# Autodesk Inventor assembly: Assembly1
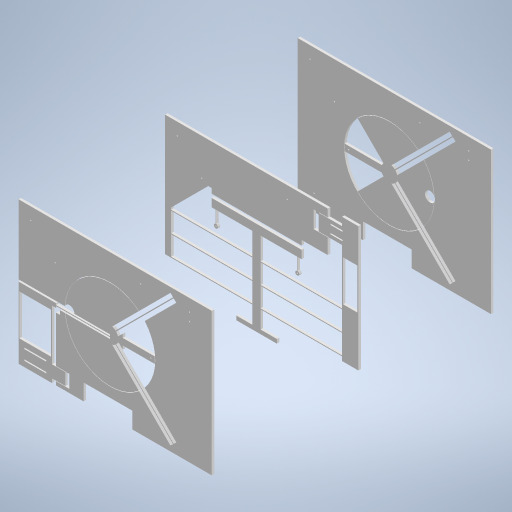
[picture p0: Inventor's stored thumbnail of the model, 512x512]
Saved by Autodesk Inventor 2023 (Build 270158000, 158)
## iProperties
Created: 2023-05-10
Part Number: Assembly1
Document SubType Name: Assembly
Designer: Nathann
Author: Nathann
## Documents named in this file (4)
- C:\Users\Nathann\OneDrive\ClawdDrive\Objet3D\IminaProbe\RoueMDF\Assembly1.iam
- C:\Users\Nathann\OneDrive\ClawdDrive\Objet3D\IminaProbe\RoueMDF\Wheel1.ipt
- C:\Users\Nathann\OneDrive\ClawdDrive\Objet3D\IminaProbe\RoueMDF\Inverter.ipt
- C:\Users\Nathann\OneDrive\ClawdDrive\Objet3D\IminaProbe\RoueMDF\Wheel2.ipt
## Components (3 placed, 3 different names)
1. Wheel1:1 — Flush:1, Flush:2, Flush:3, Flush:4, Flush:5, Flush:6, Mate:1, Mate:2
2. Inverter:1 — Flush:1, Flush:2, Flush:6
3. Wheel2:1 — Flush:3, Flush:4, Flush:5
## Relationships (8: Flush 6, Mate 2)
- Flush:1: Wheel1:1 ↔ Inverter:1
- Flush:2: Wheel1:1 ↔ Inverter:1
- Flush:3: Wheel1:1 ↔ Wheel2:1
- Flush:4: Wheel1:1 ↔ Wheel2:1
- Flush:5: Wheel1:1 ↔ Wheel2:1
- Flush:6: Wheel1:1 ↔ Inverter:1
- Mate:1: Wheel1:1
- Mate:2: Wheel1:1
